# Autodesk Inventor assembly: LEG2
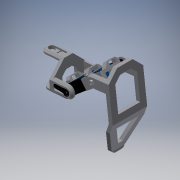
[picture p0: Inventor's stored thumbnail of the model, 180x180]
Saved by Autodesk Inventor 2017.3 (Build 213256000, 256)
## iProperties
Created: 2018-01-10
Part Number: LEG2
Document SubType Name: Assembly
Designer: Alex
Author: Alex
## Documents named in this file (9)
- X:\Alex\Documents\Git\HeRo-Mini\Hardware\LEG.iam
- X:\Alex\Documents\Git\HeRo-Mini\Hardware\FEMUR.ipt
- X:\Alex\Documents\Git\HeRo-Mini\Hardware\COXA.ipt
- X:\Alex\Documents\Git\HeRo-Mini\Hardware\SERVO.iam
- X:\Alex\Documents\Git\HeRo-Mini\Hardware\TIBIA.ipt
- X:\Alex\Documents\Git\HeRo-Mini\Hardware\M2_SCREW_8MM.ipt
- X:\Alex\Documents\Git\HeRo-Mini\Hardware\BEARING.ipt
- X:\Alex\Documents\Git\HeRo-Mini\Hardware\M3_SCREW_8MM.ipt
- X:\Alex\Documents\Git\HeRo-Mini\Hardware\NUT_3MM.ipt
## Components (15 placed, 8 different names)
1. FEMUR:1 — Rigid:1, Rigid:2, Rigid:11, Rigid:13
2. COXA:1 — Rigid:3, Rigid:9
3. SERVO:1 [sub-assembly] — Rigid:1, Rigid:3, Rigid:5, Rigid:6
4. SERVO:2 [sub-assembly] — Rigid:2, Rigid:7, Rigid:8, Rigid:15
5. TIBIA:1 — Rigid:15, Rigid:16
6. M2_SCREW_8MM:1 — Rigid:8
7. M2_SCREW_8MM:2 — Rigid:7
8. M2_SCREW_8MM:3 — Rigid:6
9. M2_SCREW_8MM:4 — Rigid:5
10. BEARING:1 — Rigid:9
11. BEARING:2 — Rigid:16
12. M3_SCREW_8MM:1 — Rigid:12
13. M3_SCREW_8MM:2 — Rigid:14
14. NUT_3MM:1 — Rigid:13, Rigid:14
15. NUT_3MM:2 — Rigid:11, Rigid:12
## Relationships (14: WeldJoint 14)
- Rigid:1 [WeldJoint]: FEMUR:1 ↔ SERVO:1
- Rigid:2 [WeldJoint]: FEMUR:1 ↔ SERVO:2
- Rigid:3 [WeldJoint]: COXA:1 ↔ SERVO:1
- Rigid:5 [WeldJoint]: SERVO:1 ↔ M2_SCREW_8MM:4
- Rigid:6 [WeldJoint]: SERVO:1 ↔ M2_SCREW_8MM:3
- Rigid:7 [WeldJoint]: SERVO:2 ↔ M2_SCREW_8MM:2
- Rigid:8 [WeldJoint]: SERVO:2 ↔ M2_SCREW_8MM:1
- Rigid:9 [WeldJoint]: COXA:1 ↔ BEARING:1
- Rigid:11 [WeldJoint]: FEMUR:1 ↔ NUT_3MM:2
- Rigid:12 [WeldJoint]: M3_SCREW_8MM:1 ↔ NUT_3MM:2
- Rigid:13 [WeldJoint]: FEMUR:1 ↔ NUT_3MM:1
- Rigid:14 [WeldJoint]: M3_SCREW_8MM:2 ↔ NUT_3MM:1
- Rigid:15 [WeldJoint]: SERVO:2 ↔ TIBIA:1
- Rigid:16 [WeldJoint]: TIBIA:1 ↔ BEARING:2
